# Autodesk Inventor assembly: Стенка БСП
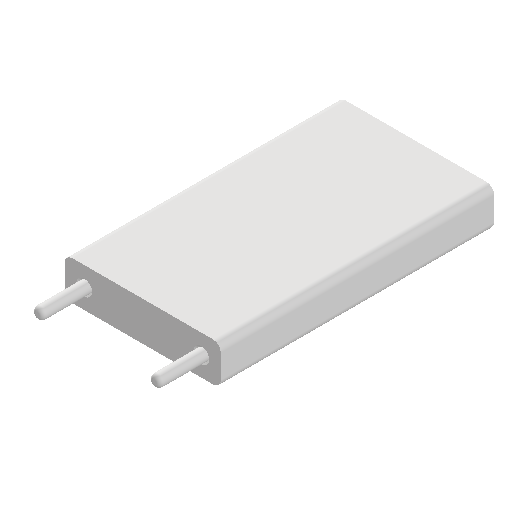
[picture p0: Inventor's stored thumbnail of the model, 512x512]
Saved by Autodesk Inventor 2022 (Build 260153000, 153)
## iProperties
Created: 2023-02-18
Part Number: Стенка БСП
Document SubType Name: Assembly
Designer: Глеб
Mass: 27.9198 g
Surface Area: 100.464 cm^2
Volume: 27.9198 cm^3
Density: 1 g/cm^3
Author: Глеб
## Documents named in this file (3)
- C:\Users\Глеб\Documents\Inventor\Файлы Inventor\Стенка БСП.iam
- C:\Users\Глеб\Documents\Inventor\Файлы Inventor\Стенка БСП.ipt
- C:\Users\Глеб\Documents\Inventor\Файлы Inventor\Шпилька крепления к несущеф стене.ipt
## Components (3 placed, 2 different names)
1. Стенка БСП:1 — Совмещение:1, Заподлицо:2, Совмещение:2, Совмещение:3
2. Шпилька крепления к несущеф стене:1 — Заподлицо:1, Совмещение:2, Совмещение:3
3. Шпилька крепления к несущеф стене:2 — Совмещение:1, Заподлицо:1, Заподлицо:2
## Relationships (5: Mate 3, Flush 2)
- Совмещение:1 [Mate]: Стенка БСП:1 ↔ Шпилька крепления к несущеф стене:2
- Заподлицо:1 [Flush]: Шпилька крепления к несущеф стене:1 ↔ Шпилька крепления к несущеф стене:2
- Заподлицо:2 [Flush] (-12 mm): Стенка БСП:1 ↔ Шпилька крепления к несущеф стене:2
- Совмещение:2 [Mate]: Стенка БСП:1 ↔ Шпилька крепления к несущеф стене:1
- Совмещение:3 [Mate]: Стенка БСП:1 ↔ Шпилька крепления к несущеф стене:1
